# Autodesk Inventor assembly: joint_assembly
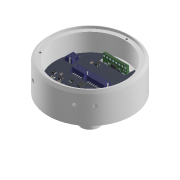
[picture p0: Inventor's stored thumbnail of the model, 180x180]
Saved by Autodesk Inventor 2017 (Build 210142000, 142)
## iProperties
Created: 2017-12-13
Part Number: joint_assembly
Document SubType Name: Assembly
Designer: Thoma
Author: Thoma
## Documents named in this file (4)
- C:\Users\Thoma\Documents\SDUEmbedded\pendulum\joint\joint_assembly.iam
- C:\Users\Thoma\Documents\SDUEmbedded\pendulum\joint_board\step\joint_board.ipt
- C:\Users\Thoma\Documents\SDUEmbedded\pendulum\joint_board\step\RLC2IC-3D.ipt
- C:\Users\Thoma\Documents\master\components\joint\joint_read_side.ipt
## Components (3 placed, 3 different names)
1. joint_board:1 — Mate:1, Angle:1, Mate:2
2. RLC2IC-3D:1 — Mate:3, Flush:1
3. joint_read_side:1 — Mate:1, Angle:1, Mate:2, Mate:3, Flush:1
## Relationships (5: Mate 3, Angle 1, Flush 1)
- Mate:1: joint_board:1 ↔ joint_read_side:1
- Angle:1 (0 deg): joint_board:1 ↔ joint_read_side:1
- Mate:2: joint_board:1 ↔ joint_read_side:1
- Mate:3: RLC2IC-3D:1 ↔ joint_read_side:1
- Flush:1 (-0.4 mm): RLC2IC-3D:1 ↔ joint_read_side:1
